# Autodesk Inventor assembly: rope_climber
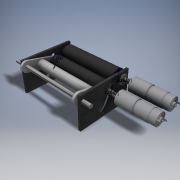
[picture p0: Inventor's stored thumbnail of the model, 180x180]
Saved by Autodesk Inventor 2017 (Build 210142000, 142)
## iProperties
Created: 2017-01-16
Part Number: rope_climber
Document SubType Name: Assembly
Designer: mmarkle
Author: mmarkle
## Documents named in this file (8)
- C:\Users\mmarkle\Documents\Robotics\Rope_Climber\Rope_Climber\rope_climber.iam
- C:\Users\mmarkle\Documents\Robotics\Rope_Climber\Rope_Climber\Roller.ipt
- C:\Users\mmarkle\Documents\Robotics\Rope_Climber\Rope_Climber\Axle.ipt
- C:\Users\mmarkle\Documents\Robotics\Rope_Climber\Rope_Climber\bearing.iam
- C:\Users\mmarkle\Documents\Robotics\Rope_Climber\Rope_Climber\toggle.ipt
- C:\Users\mmarkle\Documents\Robotics\Rope_Climber\Rope_Climber\toggle_axle.ipt
- C:\Users\mmarkle\Documents\Robotics\Rope_Climber\Rope_Climber\side_plate.ipt
- C:\Users\mmarkle\Documents\Robotics\Rope_Climber\Rope_Climber\PG-71-am-0914.ipt
## Components (14 placed, 7 different names)
1. Roller:1 — Mate:1, Mate:2
2. Roller:2 — Mate:3, Mate:4
3. Axle:1 — Mate:1, Mate:2, Mate:5, Mate:6, Mate:11, Mate:12, Mate:19, Mate:20
4. Axle:2 — Mate:3, Mate:4, Mate:7, Mate:8, Mate:9, Mate:10, Mate:17, Mate:18
5. bearing:1 [sub-assembly] — Mate:5, Mate:6, Insert:3
6. bearing:2 [sub-assembly] — Mate:7, Mate:8, Insert:1
7. bearing:3 [sub-assembly] — Mate:11, Mate:12, Insert:4
8. bearing:4 [sub-assembly] — Mate:9, Mate:10, Insert:2
9. toggle:1 — Insert:1, Insert:2, Mate:13
10. toggle_axle:1 — Mate:13, Mate:14, Mate:15
11. side_plate:1 — Insert:3, Mate:14, Angle:1, Mate:16
12. side_plate:2 — Insert:4, Mate:15, Angle:2, Mate:16
13. PG-71-am-0914:1 — Mate:19, Mate:20
14. PG-71-am-0914:2 — Mate:17, Mate:18
## Relationships (26: Mate 20, Insert 4, Angle 2)
- Mate:1: Roller:1 ↔ Axle:1
- Mate:2: Roller:1 ↔ Axle:1
- Mate:3: Roller:2 ↔ Axle:2
- Mate:4: Roller:2 ↔ Axle:2
- Mate:5: Axle:1 ↔ bearing:1
- Mate:6: Axle:1 ↔ bearing:1
- Mate:7: Axle:2 ↔ bearing:2
- Mate:8: Axle:2 ↔ bearing:2
- Mate:9: Axle:2 ↔ bearing:4
- Mate:10: Axle:2 ↔ bearing:4
- Mate:11: Axle:1 ↔ bearing:3
- Mate:12: Axle:1 ↔ bearing:3
- Insert:1: bearing:2 ↔ toggle:1
- Insert:2: bearing:4 ↔ toggle:1
- Mate:13: toggle:1 ↔ toggle_axle:1
- Insert:3: bearing:1 ↔ side_plate:1
- Insert:4: bearing:3 ↔ side_plate:2
- Mate:14: toggle_axle:1 ↔ side_plate:1
- Mate:15: toggle_axle:1 ↔ side_plate:2
- Angle:1 (0 deg): side_plate:1
- Angle:2 (180 deg): side_plate:2
- Mate:16 (228.6 mm): side_plate:1 ↔ side_plate:2
- Mate:17: Axle:2 ↔ PG-71-am-0914:2
- Mate:18: Axle:2 ↔ PG-71-am-0914:2
- Mate:19: Axle:1 ↔ PG-71-am-0914:1
- Mate:20: Axle:1 ↔ PG-71-am-0914:1
